# Autodesk Inventor assembly: Zespół1
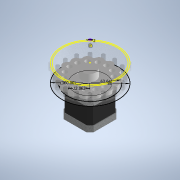
[picture p0: Inventor's stored thumbnail of the model, 180x180]
Saved by Autodesk Inventor 2021 (Build 250183000, 183)
## iProperties
Created: 2022-07-20
Part Number: Zespół1
Document SubType Name: Assembly
Designer: MicnedSQ
Author: MicnedSQ
## Documents named in this file (5)
- C:\Users\MicnedSQ\Desktop\V1\Zespół1.iam
- C:\Users\MicnedSQ\Desktop\V1\PM Wantai 609  Nema 17.ipt
- C:\Users\MicnedSQ\Desktop\V1\Joint.ipt
- C:\Users\MicnedSQ\Desktop\V1\Rotor.ipt
- C:\Users\MicnedSQ\Desktop\V1\Rotor_shaft_2.ipt
## Components (4 placed, 4 different names)
1. PM Wantai 609  Nema 17:1 — Obrotowe:1, Obrotowe:2
2. Joint:1 — Obrotowe:1
3. Rotor_shaft_2:1 — Obrotowe:2, Obrotowe:3, Obrót:1
4. Rotor:1 — Obrotowe:3, Obrót:1
## Relationships (4: RevoluteJoint 3, RelateRotation 1)
- Obrotowe:1 [RevoluteJoint]: PM Wantai 609  Nema 17:1 ↔ Joint:1
- Obrotowe:2 [RevoluteJoint]: PM Wantai 609  Nema 17:1 ↔ Rotor_shaft_2:1
- Obrotowe:3 [RevoluteJoint]: Rotor_shaft_2:1 ↔ Rotor:1
- Obrót:1 [RelateRotation] (0.0667 ul): Rotor_shaft_2:1 ↔ Rotor:1
